# Autodesk Inventor assembly: J005217
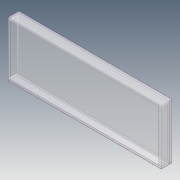
[picture p0: Inventor's stored thumbnail of the model, 180x180]
Saved by Autodesk Inventor 2015 SP1 (Build 190203100, 203)
## iProperties
Created: 2015-05-20
Vendor: HHMI: JRC - ID&F
Document SubType Name: Assembly
Designer: ARNOLDJ
Part Number: J005217
Description: MBS TROUGH ASSY
Project: P-201804
RuleStatus: InUse
AfterDocSave0: file://Part Number Cleaner
DESIGN DEPARTMENT: HHMI: JRC - ID&F
LAB/DEPT: SVOBODA (LAB)
REQUESTING SCIENTIST: SOFRONIEW, NICK
SPECIAL FINISH: NONE
SURFACE ROUGHNESS: N/A
ALTERED ITEM PART NUMBER: N/A
ALTERED ITEM VENDOR: N/A
ALTERED ITEM DESCRIPTION: N/A
Author: ARNOLDJ
Revision Number: -
## Documents named in this file (4)
- C:\_WORKSPACE\DATA\PROJECTS\MOUSE POSITIONING SYSTEM\MCAD\BALL SETUP\MBS TROUGH ASSY.iam
- C:\_WORKSPACE\DATA\PROJECTS\MOUSE POSITIONING SYSTEM\MCAD\BALL SETUP\MBS TROUGH BASE.ipt
- C:\_WORKSPACE\DATA\PROJECTS\MOUSE POSITIONING SYSTEM\MCAD\BALL SETUP\MBS TROUGH SIDE.ipt
- C:\_WORKSPACE\DATA\PROJECTS\MOUSE POSITIONING SYSTEM\MCAD\BALL SETUP\MBS TROUGH END.ipt
## Components (5 placed, 3 different names)
1. MBS TROUGH BASE:1 — Mate:1, Flush:3, Mate:2, Mate:3, Flush:4, Flush:5, Mate:4, Mate:6
2. MBS TROUGH SIDE:1 — Mate:1, Flush:3, Mate:2, Flush:6, Mate:5, Mate:7
3. MBS TROUGH SIDE:2 — Mate:3, Flush:4, Flush:5, Flush:7
4. MBS TROUGH END:1 — Mate:4, Flush:6, Mate:5
5. MBS TROUGH END:2 — Mate:6, Mate:7, Flush:7
## Relationships (12: Mate 7, Flush 5)
- Mate:1: MBS TROUGH BASE:1 ↔ MBS TROUGH SIDE:1
- Flush:3: MBS TROUGH BASE:1 ↔ MBS TROUGH SIDE:1
- Mate:2: MBS TROUGH BASE:1 ↔ MBS TROUGH SIDE:1
- Mate:3: MBS TROUGH BASE:1 ↔ MBS TROUGH SIDE:2
- Flush:4: MBS TROUGH BASE:1 ↔ MBS TROUGH SIDE:2
- Flush:5: MBS TROUGH BASE:1 ↔ MBS TROUGH SIDE:2
- Mate:4: MBS TROUGH BASE:1 ↔ MBS TROUGH END:1
- Flush:6: MBS TROUGH SIDE:1 ↔ MBS TROUGH END:1
- Mate:5: MBS TROUGH SIDE:1 ↔ MBS TROUGH END:1
- Mate:6: MBS TROUGH BASE:1 ↔ MBS TROUGH END:2
- Mate:7: MBS TROUGH SIDE:1 ↔ MBS TROUGH END:2
- Flush:7: MBS TROUGH SIDE:2 ↔ MBS TROUGH END:2
